# Autodesk Inventor assembly: bunkBedNightStand
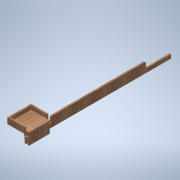
[picture p0: Inventor's stored thumbnail of the model, 180x180]
Saved by Autodesk Inventor 2021 (Build 250183000, 183)
## iProperties
Created: 2015-09-21
Part Number: bunkBedNightStand
Document SubType Name: Assembly
Designer: xdlea
Author: xdlea
## Documents named in this file (7)
- D:\OneDrive\3D Models\Bunk Bed Nightstand\bunkBedNightStand.iam
- D:\OneDrive\3D Models\Bunk Bed Nightstand\backPlate.ipt
- D:\OneDrive\3D Models\Bunk Bed Nightstand\sidePlate.ipt
- D:\OneDrive\3D Models\Bunk Bed Nightstand\topPlate.ipt
- D:\OneDrive\3D Models\Bunk Bed Nightstand\framePlate.ipt
- D:\OneDrive\3D Models\Bunk Bed Nightstand\shelfBracket.ipt
- D:\OneDrive\3D Models\Bunk Bed Nightstand\Frame.ipt
## Components (9 placed, 6 different names)
1. backPlate:1 — Mate:2, Flush:3, Flush:4, Flush:5, Mate:6
2. sidePlate:1 — Mate:3, Flush:4, Mate:6, Flush:13
3. topPlate:1 — Mate:1, Mate:2, Mate:3, Flush:6, Mate:4, Flush:7, Flush:8, Mate:5, Mate:7, Mate:15, Mate:16
4. sidePlate:2 — Mate:1, Flush:3, Flush:5, Flush:6, Flush:7, Mate:8, Flush:9
5. framePlate:1 — Mate:7, Mate:8, Flush:9, Flush:10, Flush:11, Mate:13, Mate:14, Mate:21
6. framePlate:2 — Flush:10, Flush:11, Mate:20, Flush:12
7. shelfBracket:1 — Mate:13, Mate:15, Mate:17
8. shelfBracket:2 — Mate:14, Mate:16, Mate:18
9. Frame:1 — Mate:20, Mate:21, Flush:12, Flush:13
## Relationships (27: Mate 16, Flush 11)
- Mate:1: topPlate:1 ↔ sidePlate:2
- Mate:2: backPlate:1 ↔ topPlate:1
- Mate:3: sidePlate:1 ↔ topPlate:1
- Flush:3: backPlate:1 ↔ sidePlate:2
- Flush:4: backPlate:1 ↔ sidePlate:1
- Flush:5: backPlate:1 ↔ sidePlate:2
- Flush:6 (50.8 mm): topPlate:1 ↔ sidePlate:2
- Mate:4: topPlate:1
- Flush:7: topPlate:1 ↔ sidePlate:2
- Flush:8: topPlate:1
- Mate:5: topPlate:1
- Mate:6: backPlate:1 ↔ sidePlate:1
- Mate:7: topPlate:1 ↔ framePlate:1
- Mate:8: sidePlate:2 ↔ framePlate:1
- Flush:9: sidePlate:2 ↔ framePlate:1
- Flush:10: framePlate:1 ↔ framePlate:2
- Flush:11: framePlate:1 ↔ framePlate:2
- Mate:13: framePlate:1 ↔ shelfBracket:1
- Mate:14: framePlate:1 ↔ shelfBracket:2
- Mate:15: topPlate:1 ↔ shelfBracket:1
- Mate:16: topPlate:1 ↔ shelfBracket:2
- Mate:17 (-88.9 mm): shelfBracket:1
- Mate:18 (88.9 mm): shelfBracket:2
- Mate:20: framePlate:2 ↔ Frame:1
- Mate:21: framePlate:1 ↔ Frame:1
- Flush:12: framePlate:2 ↔ Frame:1
- Flush:13: sidePlate:1 ↔ Frame:1
## Named parameters: RailHeight = 50.8 mm, Length = 266.7 mm
